# Autodesk Inventor assembly: Cable Mount
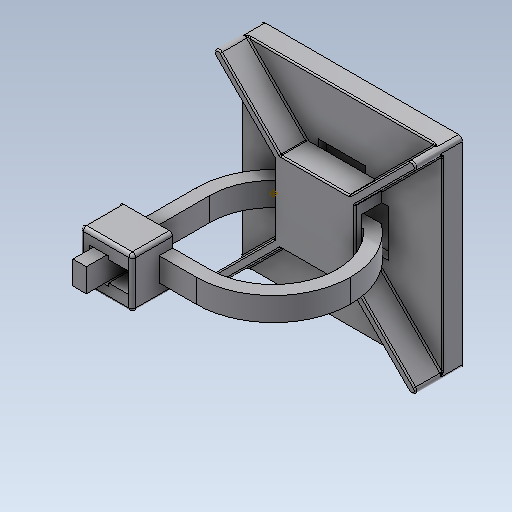
[picture p0: Inventor's stored thumbnail of the model, 512x512]
Saved by Autodesk Inventor 2020.1 (Build 241239000, 239)
## iProperties
Created: 2005-11-11
Part Number: Cable Mount
Document SubType Name: Assembly
Designer: Autodesk
Mass: 1.37832 g
Surface Area: 17.1493 cm^2
Volume: 0.984516 cm^3
Density: 1.4 g/cm^3
Total Footprint: 0.000 kg
Author: Autodesk
## Documents named in this file (3)
- C:\Users\thom_tremblay\Desktop\Inventor ACP prep data\Week 1\Electrical Enclosure\Cable Mount.iam
- C:\Users\thom_tremblay\Desktop\Inventor ACP prep data\Week 1\Electrical Enclosure\Tie wrap.ipt
- C:\Users\thom_tremblay\Desktop\Inventor ACP prep data\Week 1\Electrical Enclosure\Tie base.ipt
## Components (2 placed, 2 different names)
1. Tie base:1 — Mate:2, Angle:1, Mate:3
2. Tie wrap:1 — Mate:2, Angle:1, Mate:3
## Relationships (3: Mate 2, Angle 1)
- Mate:2: Tie base:1 ↔ Tie wrap:1
- Angle:1 (0 deg): Tie base:1 ↔ Tie wrap:1
- Mate:3: Tie base:1 ↔ Tie wrap:1
